# Autodesk Inventor assembly: Assembly
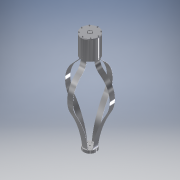
[picture p0: Inventor's stored thumbnail of the model, 180x180]
Saved by Autodesk Inventor 2017 (Build 210142000, 142)
## iProperties
Created: 2016-06-15
Part Number: Assembly
Document SubType Name: Assembly
Designer: Andres
Author: Andres
## Documents named in this file (13)
- \\Mac\Home\Documents\repositorios\BoreholeCamera\CAD_Probe\Assembly\Assembly.iam
- \\Mac\Home\Documents\repositorios\BoreholeCamera\CAD_Probe\Enclosure\Assembly\Assembly1.iam
- \\Mac\Home\Documents\repositorios\BoreholeCamera\CAD_Probe\Enclosure\Parts\91075A212_18-8 SS MALE-FEM THRDED HEX STANDOFF.ipt
- \\Mac\Home\Documents\repositorios\BoreholeCamera\CAD_Probe\Camera\Assembly\Assembly.iam
- \\Mac\Home\Documents\repositorios\BoreholeCamera\CAD_Probe\Enclosure\Parts\90910A680_LOW-PROFILE BUTTON HEAD TORX MACHINE SCREW.ipt
- \\Mac\Home\Documents\repositorios\BoreholeCamera\CAD_Probe\Enclosure\Parts\91115A816_18-8 SS FEM THRDED HEX STANDOFF.ipt
- \\Mac\Home\Documents\repositorios\BoreholeCamera\CAD_Probe\PCB\STEP\PCB_Probe.iam
- \\Mac\Home\Documents\repositorios\BoreholeCamera\CAD_Probe\Enclosure\Parts\92185A071_TYPE 316 SS SOCKET HEAD CAP SCREW.ipt
- \\Mac\Home\Documents\repositorios\BoreholeCamera\CAD_Probe\Enclosure\Parts\92785A148_HIGH HOLD CONE POINT SET SCREW.ipt
- \\Mac\Home\Documents\repositorios\BoreholeCamera\CAD_Probe\Enclosure\Parts\8inch_Fin.ipt
- \\Mac\Home\Documents\repositorios\BoreholeCamera\CAD_Probe\Enclosure\Parts\Bottom.ipt
- \\Mac\Home\Documents\repositorios\BoreholeCamera\CAD_Probe\Enclosure\Parts\92313A154_TYPE 316 SS CUP POINT SET SCREW.ipt
- \\Mac\Home\Documents\repositorios\BoreholeCamera\CAD_Probe\Enclosure\Parts\AS 568 - DASH # 004(1).ipt
## Components (42 placed, 12 different names)
1. Assembly1:1 [sub-assembly] — Insert:1, Mate:1, Insert:2, Rotation/Translation:1, Rigid:1, Rotational:1, Rotation/Translation:14, Rotation/Translation:15, Rotation/Translation:16, Rigid:2
2. 91075A212_18-8 SS MALE-FEM THRDED HEX STANDOFF:1 — Insert:1
3. 91075A212_18-8 SS MALE-FEM THRDED HEX STANDOFF:2 — Mate:1
4. 91075A212_18-8 SS MALE-FEM THRDED HEX STANDOFF:3 — Insert:2
5. 91075A212_18-8 SS MALE-FEM THRDED HEX STANDOFF:4 — Rotation/Translation:1
6. Assembly:1 [sub-assembly] — Rigid:1, Rotation/Translation:2, Rotation/Translation:3, Rotation/Translation:4, Rotation/Translation:5
7. 90910A680_LOW-PROFILE BUTTON HEAD TORX MACHINE SCREW:1 — Rotation/Translation:2
8. 90910A680_LOW-PROFILE BUTTON HEAD TORX MACHINE SCREW:2 — Rotation/Translation:3
9. 90910A680_LOW-PROFILE BUTTON HEAD TORX MACHINE SCREW:3 — Rotation/Translation:4
10. 90910A680_LOW-PROFILE BUTTON HEAD TORX MACHINE SCREW:4 — Rotation/Translation:5
11. 91115A816_18-8 SS FEM THRDED HEX STANDOFF:1 — Insert:6, Insert:9
12. 91115A816_18-8 SS FEM THRDED HEX STANDOFF:2 — Insert:5, Insert:8
13. 91115A816_18-8 SS FEM THRDED HEX STANDOFF:3 — Insert:4, Insert:7
14. 91115A816_18-8 SS FEM THRDED HEX STANDOFF:4 — Mate:2, Insert:10
15. PCB_Probe:1 [sub-assembly] — Rotational:1
16. 92185A071_TYPE 316 SS SOCKET HEAD CAP SCREW:1 — Insert:6
17. 92185A071_TYPE 316 SS SOCKET HEAD CAP SCREW:2 — Insert:5
18. 92185A071_TYPE 316 SS SOCKET HEAD CAP SCREW:3 — Insert:4
19. 92185A071_TYPE 316 SS SOCKET HEAD CAP SCREW:4 — Mate:2
20. 92785A148_HIGH HOLD CONE POINT SET SCREW:1
21. 92785A148_HIGH HOLD CONE POINT SET SCREW:2 — Rotation/Translation:14
22. 92785A148_HIGH HOLD CONE POINT SET SCREW:3 — Rotation/Translation:16
23. 92785A148_HIGH HOLD CONE POINT SET SCREW:4 — Rotation/Translation:15
24. 92185A071_TYPE 316 SS SOCKET HEAD CAP SCREW:6 — Insert:7
25. 92185A071_TYPE 316 SS SOCKET HEAD CAP SCREW:7 — Insert:8
26. 92185A071_TYPE 316 SS SOCKET HEAD CAP SCREW:8 — Insert:9
27. 92185A071_TYPE 316 SS SOCKET HEAD CAP SCREW:9 — Insert:10
28. AS 568 - DASH # 004(1):1
29. AS 568 - DASH # 004(1):2
30. Bottom:1 — Rigid:3
31. 92313A154_TYPE 316 SS CUP POINT SET SCREW:2
32. 92313A154_TYPE 316 SS CUP POINT SET SCREW:1
33. 92313A154_TYPE 316 SS CUP POINT SET SCREW:3
34. 92313A154_TYPE 316 SS CUP POINT SET SCREW:4
35. 92313A154_TYPE 316 SS CUP POINT SET SCREW:5
36. 92313A154_TYPE 316 SS CUP POINT SET SCREW:6
37. 92313A154_TYPE 316 SS CUP POINT SET SCREW:7
38. 92313A154_TYPE 316 SS CUP POINT SET SCREW:8
39. 8inch_Fin:1 — Rigid:2
40. 8inch_Fin:2 — Rigid:3
41. 8inch_Fin:3
42. 8inch_Fin:4
## Component patterns: (4 elements, first: 92313A154_TYPE 316 SS CUP POINT SET SCREW:2 + 92313A154_TYPE 316 SS CUP POINT SET SCREW:1), (4 elements, first: 8inch_Fin:1)
## Relationships (23: Insert 9, RelateRotateTranslate 8, WeldJoint 3, Mate 2, RevoluteJoint 1)
- Insert:1: Assembly1:1 ↔ 91075A212_18-8 SS MALE-FEM THRDED HEX STANDOFF:1
- Mate:1: Assembly1:1 ↔ 91075A212_18-8 SS MALE-FEM THRDED HEX STANDOFF:2
- Insert:2: Assembly1:1 ↔ 91075A212_18-8 SS MALE-FEM THRDED HEX STANDOFF:3
- Rotation/Translation:1 [RelateRotateTranslate] (4.995 mm): Assembly1:1 ↔ 91075A212_18-8 SS MALE-FEM THRDED HEX STANDOFF:4
- Rigid:1 [WeldJoint] (9.525 mm): Assembly1:1 ↔ Assembly:1
- Rotation/Translation:2 [RelateRotateTranslate] (13.087 mm): Assembly:1 ↔ 90910A680_LOW-PROFILE BUTTON HEAD TORX MACHINE SCREW:1
- Rotation/Translation:3 [RelateRotateTranslate] (13.087 mm): Assembly:1 ↔ 90910A680_LOW-PROFILE BUTTON HEAD TORX MACHINE SCREW:2
- Rotation/Translation:4 [RelateRotateTranslate] (13.087 mm): Assembly:1 ↔ 90910A680_LOW-PROFILE BUTTON HEAD TORX MACHINE SCREW:3
- Rotation/Translation:5 [RelateRotateTranslate] (13.087 mm): Assembly:1 ↔ 90910A680_LOW-PROFILE BUTTON HEAD TORX MACHINE SCREW:4
- Rotational:1 [RevoluteJoint] (23.825 mm): Assembly1:1 ↔ PCB_Probe:1
- Rotation/Translation:14 [RelateRotateTranslate] (1 mm): Assembly1:1 ↔ 92785A148_HIGH HOLD CONE POINT SET SCREW:2
- Rotation/Translation:15 [RelateRotateTranslate] (1 mm): Assembly1:1 ↔ 92785A148_HIGH HOLD CONE POINT SET SCREW:4
- Rotation/Translation:16 [RelateRotateTranslate] (1 mm): Assembly1:1 ↔ 92785A148_HIGH HOLD CONE POINT SET SCREW:3
- Insert:4 (0.4115 mm): 91115A816_18-8 SS FEM THRDED HEX STANDOFF:3 ↔ 92185A071_TYPE 316 SS SOCKET HEAD CAP SCREW:3
- Insert:5 (0.4115 mm): 91115A816_18-8 SS FEM THRDED HEX STANDOFF:2 ↔ 92185A071_TYPE 316 SS SOCKET HEAD CAP SCREW:2
- Insert:6 (0.4115 mm): 91115A816_18-8 SS FEM THRDED HEX STANDOFF:1 ↔ 92185A071_TYPE 316 SS SOCKET HEAD CAP SCREW:1
- Mate:2 (0.4115 mm): 91115A816_18-8 SS FEM THRDED HEX STANDOFF:4 ↔ 92185A071_TYPE 316 SS SOCKET HEAD CAP SCREW:4
- Insert:7 (1.6 mm): 91115A816_18-8 SS FEM THRDED HEX STANDOFF:3 ↔ 92185A071_TYPE 316 SS SOCKET HEAD CAP SCREW:6
- Insert:8 (1.6 mm): 91115A816_18-8 SS FEM THRDED HEX STANDOFF:2 ↔ 92185A071_TYPE 316 SS SOCKET HEAD CAP SCREW:7
- Insert:9 (1.6 mm): 91115A816_18-8 SS FEM THRDED HEX STANDOFF:1 ↔ 92185A071_TYPE 316 SS SOCKET HEAD CAP SCREW:8
- Insert:10 (1.6 mm): 91115A816_18-8 SS FEM THRDED HEX STANDOFF:4 ↔ 92185A071_TYPE 316 SS SOCKET HEAD CAP SCREW:9
- Rigid:2 [WeldJoint]: Assembly1:1 ↔ 8inch_Fin:1
- Rigid:3 [WeldJoint]: Bottom:1 ↔ 8inch_Fin:2
